# Autodesk Inventor assembly: FINAL_Assembly
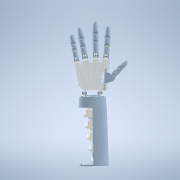
[picture p0: Inventor's stored thumbnail of the model, 180x180]
Saved by Autodesk Inventor 2022 (Build 260153000, 153)
## iProperties
Created: 2023-01-15
Part Number: FINAL_Assembly
Document SubType Name: Assembly
Designer: 48735
Author: 48735
## Documents named in this file (30)
- C:\Users\48735\Desktop\Robot_hand_CAD\OSTATECZNA WERSJA\FINAL_Assembly.iam
- C:\Users\48735\Desktop\Robot_hand_CAD\OSTATECZNA WERSJA\Main_part_hand.ipt
- C:\Users\48735\Desktop\Robot_hand_CAD\OSTATECZNA WERSJA\Thumb_assembly.iam
- C:\Users\48735\Desktop\Robot_hand_CAD\OSTATECZNA WERSJA\Index_1.ipt
- C:\Users\48735\Desktop\Robot_hand_CAD\OSTATECZNA WERSJA\Middle_1.ipt
- C:\Users\48735\Desktop\Robot_hand_CAD\OSTATECZNA WERSJA\Ring_1.ipt
- C:\Users\48735\Desktop\Robot_hand_CAD\OSTATECZNA WERSJA\Index_2.ipt
- C:\Users\48735\Desktop\Robot_hand_CAD\OSTATECZNA WERSJA\Index_3.ipt
- C:\Users\48735\Desktop\Robot_hand_CAD\OSTATECZNA WERSJA\Middle_2.ipt
- C:\Users\48735\Desktop\Robot_hand_CAD\OSTATECZNA WERSJA\Ring_2.ipt
- C:\Users\48735\Desktop\Robot_hand_CAD\OSTATECZNA WERSJA\Middle_3.ipt
- C:\Users\48735\Desktop\Robot_hand_CAD\OSTATECZNA WERSJA\Ring_3.ipt
- C:\Users\48735\Desktop\Robot_hand_CAD\OSTATECZNA WERSJA\Lil_1.ipt
- C:\Users\48735\Desktop\Robot_hand_CAD\OSTATECZNA WERSJA\Lil_2.ipt
- C:\Users\48735\Desktop\Robot_hand_CAD\OSTATECZNA WERSJA\Lil_3.ipt
- C:\Users\48735\Desktop\Robot_hand_CAD\OSTATECZNA WERSJA\Forearm_1.ipt
- C:\Users\48735\Desktop\Robot_hand_CAD\OSTATECZNA WERSJA\Wrist_1V1.ipt
- C:\Users\48735\Desktop\Robot_hand_CAD\OSTATECZNA WERSJA\ServoMotor .iam
- C:\Users\48735\Desktop\Robot_hand_CAD\OSTATECZNA WERSJA\Forearm_2.ipt
- C:\Users\48735\Desktop\Robot_hand_CAD\OSTATECZNA WERSJA\Forearm_3.ipt
- C:\Users\48735\Desktop\Robot_hand_CAD\OSTATECZNA WERSJA\Forearm_4.ipt
- C:\Users\48735\Desktop\Robot_hand_CAD\OSTATECZNA WERSJA\Connector_1.ipt
- C:\Users\48735\Desktop\Robot_hand_CAD\OSTATECZNA WERSJA\Connector_2.ipt
- C:\Users\48735\Desktop\Robot_hand_CAD\OSTATECZNA WERSJA\Connector_3.ipt
- C:\Users\48735\Documents\Inventor\Content Center Files\R2022\en-US\BS EN 24035\ISO 4035 - M5BS EN.ipt
- C:\Users\48735\Documents\Inventor\Content Center Files\R2022\en-US\CNS 4557\CNS 4557 - M5 x 0,8 x 10.ipt
- C:\Users\48735\Documents\Inventor\Content Center Files\R2022\en-US\UNI 5923\UNI 5923 - M3 x 16 - 0,5.ipt
- C:\Users\48735\Documents\Inventor\Content Center Files\R2022\en-US\UNI 5923\UNI 5923 - M3 x 14 - 0,5.ipt
- C:\Users\48735\Desktop\Robot_hand_CAD\OSTATECZNA WERSJA\Spring_hand.ipt
- C:\Users\48735\Desktop\Robot_hand_CAD\OSTATECZNA WERSJA\Spring_thumb.ipt
## Components (81 placed, 29 different names)
1. Main_part_hand:1 — Rotational:1, Rotational:2, Rotational:3, Rotational:4, Rotational:11, Rotational:19, Insert:15, Insert:16, Rotational:20, Rotational:21, Rotational:22, Rotational:23, Rotational:24, Rotational:25, Rotational:26, Rotational:27, Rigid:47
2. Thumb_assembly:1 [sub-assembly] — Rotational:1, Rigid:45, Rigid:46
3. Index_1:1 — Rotational:2, Rotational:5, Rigid:33, Rigid:34
4. Middle_1:1 — Rotational:3, Rotational:12, Rigid:36, Rigid:37
5. Ring_1:1 — Rotational:4, Rotational:13, Rigid:39, Rigid:40
6. Index_2:1 — Rotational:5, Rotational:6, Rigid:35, Rotational:31, Rotational:35
7. Index_3:1 — Rotational:6, Rotational:39, Rotational:40
8. Middle_2:1 — Rotational:12, Rotational:17, Rigid:38, Rotational:30, Rotational:34
9. Ring_2:1 — Rotational:13, Rotational:16, Rigid:41, Rotational:29, Rotational:33
10. Middle_3:1 — Rotational:17, Rotational:38, Rotational:41
11. Ring_3:1 — Rotational:16, Rotational:37, Rotational:42
12. Lil_1:1 — Rotational:11, Rotational:14, Rigid:42, Rigid:43
13. Lil_2:1 — Rotational:14, Rotational:15, Rigid:44, Rotational:28, Rotational:32
14. Lil_3:1 — Rotational:15, Rotational:36, Rotational:43
15. Wrist_1V1:1 — Rigid:29, Rigid:31, Rigid:32, Rigid:47
16. Forearm_1:1 — Rigid:27, Rigid:26, Rigid:25, Rigid:24, Rigid:23, Rigid:28, Insert:5
17. ServoMotor :1 [sub-assembly] — Rigid:23, Insert:13, Insert:14
18. ServoMotor :2 [sub-assembly] — Rigid:25, Insert:9, Insert:10
19. ServoMotor :3 [sub-assembly] — Rigid:27, Insert:6
20. ServoMotor :4 [sub-assembly] — Rigid:26, Insert:7, Insert:8
21. ServoMotor :5 [sub-assembly] — Rigid:24, Insert:11, Insert:12
22. Forearm_2:1 — Rigid:28, Rigid:29, Rigid:30, Rotational:18, Insert:1, Insert:2, Insert:3
23. Forearm_3:1 — Rigid:30
24. Forearm_4:1 — Rotational:18, Insert:4
25. Connector_1:1 — Rotational:19
26. Connector_2:1 — Insert:2
27. Connector_2:2 — Insert:1
28. Connector_2:3 — Insert:4
29. Connector_2:4 — Insert:3
30. Connector_3:1 — Insert:14
31. Connector_3:2 — Insert:13
32. Connector_3:3 — Insert:12
33. Connector_3:4 — Insert:11
34. Connector_3:5 — Insert:10
35. Connector_3:6 — Insert:9
36. Connector_3:7 — Insert:8
37. Connector_3:8 — Insert:7
38. Connector_3:9 — Insert:6
39. Connector_3:10 — Insert:5
40. BS EN 24035 - Metric M5:1 — Rigid:31
41. BS EN 24035 - Metric M5:2 — Rigid:32
42. CNS 4557 M5 x 10:1 — Insert:16
43. CNS 4557 M5 x 10:2 — Insert:15
44. UNI 5923 M3 x 16:1 — Rigid:41
45. UNI 5923 M3 x 16:2 — Rigid:40
46. UNI 5923 M3 x 16:3 — Rigid:39
47. UNI 5923 M3 x 16:4 — Rigid:35
48. UNI 5923 M3 x 16:5 — Rigid:36
49. UNI 5923 M3 x 16:6 — Rigid:33
50. UNI 5923 M3 x 16:7 — Rigid:38
51. UNI 5923 M3 x 16:8 — Rigid:37
52. UNI 5923 M3 x 16:9 — Rigid:34
53. UNI 5923 M3 x 14:1 — Rigid:42
54. UNI 5923 M3 x 14:2 — Rigid:43
55. UNI 5923 M3 x 14:3 — Rigid:44
56. UNI 5923 M3 x 14:4 — Rigid:45
57. UNI 5923 M3 x 14:5 — Rigid:46
58. Spring_hand:1 — Rotational:20
59. Spring_hand:2 — Rotational:21
60. Spring_hand:3 — Rotational:22
61. Spring_hand:4 — Rotational:23
62. Spring_hand:5 — Rotational:25
63. Spring_hand:6 — Rotational:24
64. Spring_thumb:1 — Rotational:28
65. Spring_thumb:2 — Rotational:27
66. Spring_thumb:3 — Rotational:26
67. Spring_thumb:4 — Rotational:29
68. Spring_thumb:5 — Rotational:30
69. Spring_thumb:6 — Rotational:31
70. Spring_thumb:7 — Rotational:33
71. Spring_thumb:8 — Rotational:38
72. Spring_thumb:9 — Rotational:39
73. Spring_thumb:10 — Rotational:32
74. Spring_thumb:11 — Rotational:34
75. Spring_thumb:12 — Rotational:35
76. Spring_thumb:13 — Rotational:36
77. Spring_thumb:14 — Rotational:37
78. Spring_thumb:15 — Rotational:40
79. Spring_thumb:16 — Rotational:41
80. Spring_thumb:17 — Rotational:42
81. Spring_thumb:18 — Rotational:43
## Relationships (80: RevoluteJoint 39, WeldJoint 25, Insert 16)
- Rotational:1 [RevoluteJoint] (-0.5 mm): Main_part_hand:1 ↔ Thumb_assembly:1
- Rotational:2 [RevoluteJoint]: Main_part_hand:1 ↔ Index_1:1
- Rotational:3 [RevoluteJoint]: Main_part_hand:1 ↔ Middle_1:1
- Rotational:4 [RevoluteJoint]: Main_part_hand:1 ↔ Ring_1:1
- Rotational:5 [RevoluteJoint]: Index_1:1 ↔ Index_2:1
- Rotational:6 [RevoluteJoint]: Index_2:1 ↔ Index_3:1
- Rotational:11 [RevoluteJoint]: Main_part_hand:1 ↔ Lil_1:1
- Rotational:12 [RevoluteJoint]: Middle_1:1 ↔ Middle_2:1
- Rotational:13 [RevoluteJoint]: Ring_1:1 ↔ Ring_2:1
- Rotational:14 [RevoluteJoint]: Lil_1:1 ↔ Lil_2:1
- Rotational:15 [RevoluteJoint]: Lil_2:1 ↔ Lil_3:1
- Rotational:16 [RevoluteJoint]: Ring_2:1 ↔ Ring_3:1
- Rotational:17 [RevoluteJoint]: Middle_2:1 ↔ Middle_3:1
- Rigid:27 [WeldJoint]: Forearm_1:1 ↔ ServoMotor :3
- Rigid:26 [WeldJoint]: Forearm_1:1 ↔ ServoMotor :4
- Rigid:25 [WeldJoint]: Forearm_1:1 ↔ ServoMotor :2
- Rigid:24 [WeldJoint]: Forearm_1:1 ↔ ServoMotor :5
- Rigid:23 [WeldJoint]: Forearm_1:1 ↔ ServoMotor :1
- Rigid:28 [WeldJoint]: Forearm_1:1 ↔ Forearm_2:1
- Rigid:29 [WeldJoint]: Wrist_1V1:1 ↔ Forearm_2:1
- Rigid:30 [WeldJoint]: Forearm_2:1 ↔ Forearm_3:1
- Rotational:18 [RevoluteJoint]: Forearm_2:1 ↔ Forearm_4:1
- Rotational:19 [RevoluteJoint]: Main_part_hand:1 ↔ Connector_1:1
- Insert:1: Forearm_2:1 ↔ Connector_2:2
- Insert:2: Forearm_2:1 ↔ Connector_2:1
- Insert:3: Forearm_2:1 ↔ Connector_2:4
- Insert:4: Forearm_4:1 ↔ Connector_2:3
- Insert:5: Forearm_1:1 ↔ Connector_3:10
- Insert:6: ServoMotor :3 ↔ Connector_3:9
- Insert:7: ServoMotor :4 ↔ Connector_3:8
- Insert:8: ServoMotor :4 ↔ Connector_3:7
- Insert:9: ServoMotor :2 ↔ Connector_3:6
- Insert:10: ServoMotor :2 ↔ Connector_3:5
- Insert:11: ServoMotor :5 ↔ Connector_3:4
- Insert:12: ServoMotor :5 ↔ Connector_3:3
- Insert:13: ServoMotor :1 ↔ Connector_3:2
- Insert:14: ServoMotor :1 ↔ Connector_3:1
- Rigid:31 [WeldJoint]: Wrist_1V1:1 ↔ BS EN 24035 - Metric M5:1
- Rigid:32 [WeldJoint]: Wrist_1V1:1 ↔ BS EN 24035 - Metric M5:2
- Insert:15: Main_part_hand:1 ↔ CNS 4557 M5 x 10:2
- Insert:16: Main_part_hand:1 ↔ CNS 4557 M5 x 10:1
- Rigid:33 [WeldJoint] (-1 mm): Index_1:1 ↔ UNI 5923 M3 x 16:6
- Rigid:34 [WeldJoint] (-1 mm): Index_1:1 ↔ UNI 5923 M3 x 16:9
- Rigid:35 [WeldJoint] (-1 mm): Index_2:1 ↔ UNI 5923 M3 x 16:4
- Rigid:36 [WeldJoint] (-1 mm): Middle_1:1 ↔ UNI 5923 M3 x 16:5
- Rigid:37 [WeldJoint] (-1 mm): Middle_1:1 ↔ UNI 5923 M3 x 16:8
- Rigid:38 [WeldJoint] (-1 mm): Middle_2:1 ↔ UNI 5923 M3 x 16:7
- Rigid:39 [WeldJoint] (-1 mm): Ring_1:1 ↔ UNI 5923 M3 x 16:3
- Rigid:40 [WeldJoint] (-1 mm): Ring_1:1 ↔ UNI 5923 M3 x 16:2
- Rigid:41 [WeldJoint] (-1 mm): Ring_2:1 ↔ UNI 5923 M3 x 16:1
- Rigid:42 [WeldJoint] (-1 mm): Lil_1:1 ↔ UNI 5923 M3 x 14:1
- Rigid:43 [WeldJoint] (-1 mm): Lil_1:1 ↔ UNI 5923 M3 x 14:2
- Rigid:44 [WeldJoint] (-1 mm): Lil_2:1 ↔ UNI 5923 M3 x 14:3
- Rigid:45 [WeldJoint] (-1 mm): Thumb_assembly:1 ↔ UNI 5923 M3 x 14:4
- Rigid:46 [WeldJoint] (-1 mm): Thumb_assembly:1 ↔ UNI 5923 M3 x 14:5
- Rotational:20 [RevoluteJoint] (3.75 mm): Main_part_hand:1 ↔ Spring_hand:1
- Rotational:21 [RevoluteJoint]: Main_part_hand:1 ↔ Spring_hand:2
- Rotational:22 [RevoluteJoint]: Main_part_hand:1 ↔ Spring_hand:3
- Rotational:23 [RevoluteJoint] (3.75 mm): Main_part_hand:1 ↔ Spring_hand:4
- Rotational:24 [RevoluteJoint] (3.75 mm): Main_part_hand:1 ↔ Spring_hand:6
- Rotational:25 [RevoluteJoint]: Main_part_hand:1 ↔ Spring_hand:5
- Rotational:26 [RevoluteJoint]: Main_part_hand:1 ↔ Spring_thumb:3
- Rotational:27 [RevoluteJoint] (3 mm): Main_part_hand:1 ↔ Spring_thumb:2
- Rotational:28 [RevoluteJoint]: Lil_2:1 ↔ Spring_thumb:1
- Rotational:29 [RevoluteJoint]: Ring_2:1 ↔ Spring_thumb:4
- Rotational:30 [RevoluteJoint]: Middle_2:1 ↔ Spring_thumb:5
- Rotational:31 [RevoluteJoint]: Index_2:1 ↔ Spring_thumb:6
- Rotational:32 [RevoluteJoint] (3 mm): Lil_2:1 ↔ Spring_thumb:10
- Rotational:33 [RevoluteJoint] (3 mm): Ring_2:1 ↔ Spring_thumb:7
- Rotational:34 [RevoluteJoint] (3 mm): Middle_2:1 ↔ Spring_thumb:11
- Rotational:35 [RevoluteJoint] (3 mm): Index_2:1 ↔ Spring_thumb:12
- Rotational:36 [RevoluteJoint] (3 mm): Lil_3:1 ↔ Spring_thumb:13
- Rotational:37 [RevoluteJoint] (3 mm): Ring_3:1 ↔ Spring_thumb:14
- Rotational:38 [RevoluteJoint] (3 mm): Middle_3:1 ↔ Spring_thumb:8
- Rotational:39 [RevoluteJoint] (3 mm): Index_3:1 ↔ Spring_thumb:9
- Rotational:40 [RevoluteJoint]: Index_3:1 ↔ Spring_thumb:15
- Rotational:41 [RevoluteJoint]: Middle_3:1 ↔ Spring_thumb:16
- Rotational:42 [RevoluteJoint]: Ring_3:1 ↔ Spring_thumb:17
- Rotational:43 [RevoluteJoint]: Lil_3:1 ↔ Spring_thumb:18
- Rigid:47 [WeldJoint]: Main_part_hand:1 ↔ Wrist_1V1:1
